# Autodesk Inventor assembly: Robô24 v1
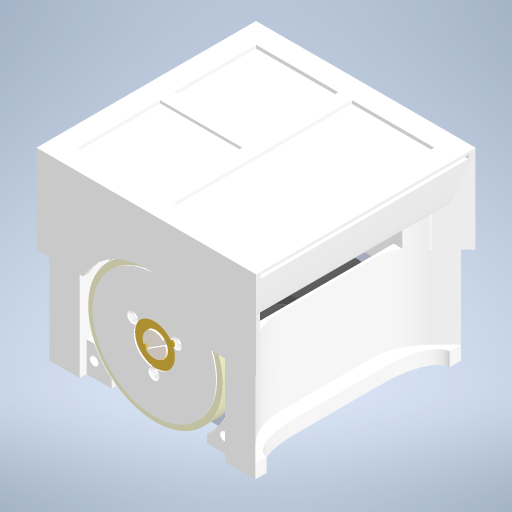
[picture p0: Inventor's stored thumbnail of the model, 512x512]
Saved by Autodesk Inventor 2024 (Build 280153000, 153)
## iProperties
Created: 2024-04-10
Part Number: Robô24 v1
Document SubType Name: Assembly
Designer: pedro
Author: pedro
## Documents named in this file (6)
- D:\pedro\Downloads\VSS 24\Robô24 v1.iam
- D:\pedro\Downloads\VSS 24\base_2024.ipt
- D:\pedro\Downloads\VSS 24\Uniform 2024.ipt
- D:\pedro\Downloads\vss-faulhaber-mechanics-master\vss-faulhaber-mechanics-master\VSS V3.0\Solidworks\Power Unit\Left_power_set\Left_power_set.ipt
- D:\pedro\Downloads\vss-faulhaber-mechanics-master\vss-faulhaber-mechanics-master\VSS V3.0\Solidworks\Power Unit\Right_power_set\Right_power_set.ipt
- D:\pedro\Downloads\vss-faulhaber-mechanics-master\vss-faulhaber-mechanics-master\VSS V3.0\Solidworks\Power Unit\Roda VSS_2022\Roda VSS_2022.ipt
## Components (6 placed, 5 different names)
1. base_2024:1 — Coincidente:1, Coincidente:2, Coincidente:3, Coincidente:4, Rotativa:1, Rígida:1
2. Uniform 2024:1 — Rotativa:1, Rígida:1
3. Left_power_set:1 — Coincidente:3, Coincidente:4, Coincidente:6
4. Right_power_set:1 — Coincidente:1, Coincidente:2, Coincidente:5
5. Roda VSS_2022:1 — Coincidente:6
6. Roda VSS_2022:2 — Coincidente:5
## Relationships (8: Mate 6, RevoluteJoint 1, WeldJoint 1)
- Coincidente:1 [Mate]: base_2024:1 ↔ Right_power_set:1
- Coincidente:2 [Mate]: base_2024:1 ↔ Right_power_set:1
- Coincidente:3 [Mate]: base_2024:1 ↔ Left_power_set:1
- Coincidente:4 [Mate]: base_2024:1 ↔ Left_power_set:1
- Coincidente:5 [Mate]: Right_power_set:1 ↔ Roda VSS_2022:2
- Coincidente:6 [Mate]: Left_power_set:1 ↔ Roda VSS_2022:1
- Rotativa:1 [RevoluteJoint]: base_2024:1 ↔ Uniform 2024:1
- Rígida:1 [WeldJoint]: base_2024:1 ↔ Uniform 2024:1
